# Autodesk Inventor assembly: Платформа_сборка - новая
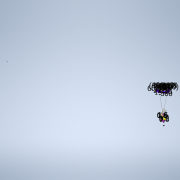
[picture p0: Inventor's stored thumbnail of the model, 180x180]
Saved by Autodesk Inventor 2020 (Build 240168000, 168)
## iProperties
Created: 2022-02-23
Part Number: Платформа_сборка - новая
Document SubType Name: Assembly
Designer: Dell
Author: Dell
## Documents named in this file (24)
- C:\Users\air13\Documents\3D\уборка\Face 2.0 full\2\Платформа_сборка - новая.iam
- C:\Users\air13\Documents\OnStage\20.05\Smile20.05VLI\Платформа_сборка_Женя\Нижний_круг_платформа.ipt
- C:\Users\air13\Documents\OnStage\20.05\Smile20.05VLI\Платформа_сборка_Женя\Крепление_мотора1_платформа.ipt
- C:\Users\air13\Documents\OnStage\20.05\Smile20.05VLI\Платформа_сборка_Женя\Крепление_мотора2_платформа.ipt
- C:\Users\air13\Documents\OnStage\20.05\Smile20.05VLI\Платформа_сборка_Женя\Крепление_мотора3_платформа.ipt
- C:\Users\air13\Documents\OnStage\20.05\Smile20.05VLI\Второй этаж\Разметка новых деталей на I этаже.ipt
- C:\Users\air13\Documents\OnStage\20.05\Smile20.05VLI\Второй этаж\Верхняя платформа.ipt
- C:\Users\air13\Documents\OnStage\20.05\Smile20.05VLI\Второй этаж\Боковой профиль.ipt
- C:\Users\air13\Documents\OnStage\20.05\Smile20.05VLI\Второй этаж\Задний профиль.ipt
- C:\Users\air13\Documents\3D\уборка\Face 2.0 full\2\шея2,0.ipt
- C:\Users\air13\Documents\OnStage\Крепление для мотора.ipt
- C:\Users\air13\Documents\OnStage\Механизм поднятия ботинка\Мотор Gekko MR25-098 без оси.ipt
- C:\Users\air13\Documents\OnStage\Механизм поднятия ботинка\Ось мотора Gekko MR25-098.ipt
- C:\Users\air13\Documents\OnStage\Механизм поднятия ботинка\Диск_для ботинка.ipt
- C:\Users\air13\Documents\OnStage\Механизм поднятия ботинка\Подшипник 604z.ipt
- C:\Users\air13\Documents\OnStage\Механизм поднятия ботинка\Поднимающая балка.ipt
- C:\Users\air13\Documents\OnStage\Механизм поднятия ботинка\Крепление_на мотор_для_диска_для ботинок.ipt
- C:\Users\air13\Documents\OnStage\Механизм поднятия ботинка\Крепление для_мотора_для руки.ipt
- C:\Users\air13\Documents\OnStage\Модель_движителя_марионеточной_опоры\Шестерня_small — копия.ipt
- C:\Users\air13\Documents\OnStage\Модель_движителя_марионеточной_опоры\Шестерня_small.ipt
- C:\Users\air13\Documents\OnStage\Модель_движителя_марионеточной_опоры\Паз_прямой_квадрат.ipt
- C:\Users\air13\Documents\OnStage\Модель_движителя_марионеточной_опоры\Шестерня_vРРО.ipt
- C:\Users\air13\Documents\OnStage\Модель_движителя_марионеточной_опоры\Проставка.ipt
- C:\Users\air13\Documents\3D\уборка\Face 2.0 full\2\ПереПереСборка лица.iam
## Components (35 placed, 22 different names)
1. Нижний_круг_платформа:1 — Угол:1, Заподлицо:1, Совмещение:1, Совмещение:2, Совмещение:3, Совмещение:5, Заподлицо:3, Совмещение:6, Заподлицо:4, Заподлицо:5, Заподлицо:6, Угол:2, Совмещение:11, Угол:3, Угол:4, Касательность:1, Совмещение:21, Совмещение:22, Совмещение:23
2. Разметка новых деталей на I этаже:1
3. Верхняя платформа:1 — Совмещение:7, Угол:2, Совмещение:8, Совмещение:9, Заподлицо:7, Совмещение:24, Совмещение:25, Угол:5, Совмещение:40, Совмещение:41, Совмещение:42, Угол:6, Совмещение:46, Совмещение:47, Совмещение:48, Совмещение:51, Совмещение:52, Совмещение:53, Совмещение:55
4. Боковой профиль:1 — Совмещение:11, Совмещение:18, Совмещение:19, Заподлицо:7, Совмещение:31
5. шея2,0:1 — Угол:3, Совмещение:13, Совмещение:19, Касательность:2, Совмещение:23, Совмещение:31, Совмещение:59, Совмещение:60
6. Задний профиль:1 — Касательность:2, Совмещение:20, Совмещение:21, Совмещение:22
7. Крепление для мотора:1 — Совмещение:24, Совмещение:25, Угол:5, Совмещение:26
8. Мотор Gekko MR25-098 без оси:1 — Совмещение:26, С поворотом:1
9. Ось мотора Gekko MR25-098:1 — С поворотом:1, С поворотом:3
10. Диск_для ботинка:1 — Совмещение:27, С поворотом:4, Совмещение:30
11. Поднимающая балка:1 — Совмещение:28, Заподлицо:8
12. Крепление_на мотор_для_диска_для ботинок:1 — С поворотом:3, Совмещение:27, Совмещение:30
13. Подшипник 604z:1 — С поворотом:4, Совмещение:28, Заподлицо:8
14. Крепление для мотора:2 — Цилиндрический:1, Совмещение:47, Совмещение:48, Совмещение:54
15. Мотор Gekko MR25-098 без оси:2 — Цилиндрический:1, С поворотом:5
16. Цилиндрическое зубчатое зацепление2:1 — Совмещение:35, Совмещение:36, Совмещение:37, Совмещение:38, Совмещение:39, Совмещение:45, Совмещение:46
17. Цилиндрическое зубчатое зацепление2:2 — Совмещение:38, Совмещение:39, Совмещение:45
18. Крепление для_мотора_для руки:1 — Цилиндрический:2, Совмещение:35, Совмещение:36, Совмещение:37
19. Ось мотора Gekko MR25-098:2 — С поворотом:5, Цилиндрический:2
20. Паз_прямой_квадрат:1 — Совмещение:40, Совмещение:41, Совмещение:42, Совмещение:43, Совмещение:44
21. Шестерня_vРРО:1 — Угол:6, Совмещение:43, Совмещение:44
22. Проставка:1 — Совмещение:51, Совмещение:52, Совмещение:53, Совмещение:54, Совмещение:55
23. ПереПереСборка лица:1 [sub-assembly] — Совмещение:59, Совмещение:60
24. Крепление_мотора1_платформа:1
25. Крепление_мотора1_платформа:2
26. Крепление_мотора1_платформа:3 — Угол:1, Заподлицо:1, Совмещение:1, Совмещение:2, Совмещение:4, Заподлицо:2
27. Крепление_мотора1_платформа:4
28. Крепление_мотора2_платформа:1 — Совмещение:5, Заподлицо:3, Совмещение:6
29. Крепление_мотора2_платформа:2
30. Крепление_мотора2_платформа:3
31. Крепление_мотора2_платформа:4
32. Крепление_мотора3_платформа:1 — Совмещение:3, Совмещение:4, Заподлицо:2
33. Крепление_мотора3_платформа:2
34. Крепление_мотора3_платформа:3
35. Крепление_мотора3_платформа:4
## Component patterns: (4 elements, first: Крепление_мотора1_платформа:1), (4 elements, first: Крепление_мотора2_платформа:1), (4 elements, first: Крепление_мотора3_платформа:1)
## Relationships (67: Mate 45, Flush 8, Angle 6, RevoluteJoint 4, Tangent 2, CylindricalJoint 2)
- Угол:1 [Angle] (0 deg): Нижний_круг_платформа:1 ↔ Крепление_мотора1_платформа:3
- Заподлицо:1 [Flush]: Нижний_круг_платформа:1 ↔ Крепление_мотора1_платформа:3
- Совмещение:1 [Mate]: Нижний_круг_платформа:1 ↔ Крепление_мотора1_платформа:3
- Совмещение:2 [Mate]: Нижний_круг_платформа:1 ↔ Крепление_мотора1_платформа:3
- Совмещение:3 [Mate]: Нижний_круг_платформа:1 ↔ Крепление_мотора3_платформа:1
- Совмещение:4 [Mate]: Крепление_мотора1_платформа:3 ↔ Крепление_мотора3_платформа:1
- Заподлицо:2 [Flush]: Крепление_мотора1_платформа:3 ↔ Крепление_мотора3_платформа:1
- Совмещение:5 [Mate]: Нижний_круг_платформа:1 ↔ Крепление_мотора2_платформа:1
- Заподлицо:3 [Flush]: Нижний_круг_платформа:1 ↔ Крепление_мотора2_платформа:1
- Совмещение:6 [Mate]: Нижний_круг_платформа:1 ↔ Крепление_мотора2_платформа:1
- Заподлицо:4 [Flush]: Нижний_круг_платформа:1
- Заподлицо:5 [Flush]: Нижний_круг_платформа:1
- Заподлицо:6 [Flush]: Нижний_круг_платформа:1
- Совмещение:7 [Mate]: Верхняя платформа:1
- Угол:2 [Angle] (0 deg): Нижний_круг_платформа:1 ↔ Верхняя платформа:1
- Совмещение:8 [Mate]: Верхняя платформа:1
- Совмещение:9 [Mate]: Верхняя платформа:1
- Совмещение:11 [Mate]: Нижний_круг_платформа:1 ↔ Боковой профиль:1
- Угол:3 [Angle] (180 deg): Нижний_круг_платформа:1 ↔ шея2,0:1
- Совмещение:13 [Mate]: шея2,0:1
- Угол:4 [Angle] (0 deg): Нижний_круг_платформа:1
- Касательность:1 [Tangent]: Нижний_круг_платформа:1
- Совмещение:18 [Mate]: Боковой профиль:1
- Совмещение:19 [Mate]: Боковой профиль:1 ↔ шея2,0:1
- Заподлицо:7 [Flush]: Верхняя платформа:1 ↔ Боковой профиль:1
- Касательность:2 [Tangent]: шея2,0:1 ↔ Задний профиль:1
- Совмещение:20 [Mate]: Задний профиль:1
- Совмещение:21 [Mate]: Нижний_круг_платформа:1 ↔ Задний профиль:1
- Совмещение:22 [Mate]: Нижний_круг_платформа:1 ↔ Задний профиль:1
- Совмещение:23 [Mate] (1035 mm): Нижний_круг_платформа:1 ↔ шея2,0:1
- Совмещение:24 [Mate]: Верхняя платформа:1 ↔ Крепление для мотора:1
- Совмещение:25 [Mate]: Верхняя платформа:1 ↔ Крепление для мотора:1
- Угол:5 [Angle] (0 deg): Верхняя платформа:1 ↔ Крепление для мотора:1
- Совмещение:26 [Mate]: Крепление для мотора:1 ↔ Мотор Gekko MR25-098 без оси:1
- С поворотом:1 [RevoluteJoint]: Мотор Gekko MR25-098 без оси:1 ↔ Ось мотора Gekko MR25-098:1
- С поворотом:3 [RevoluteJoint]: Ось мотора Gekko MR25-098:1 ↔ Крепление_на мотор_для_диска_для ботинок:1
- Совмещение:27 [Mate]: Диск_для ботинка:1 ↔ Крепление_на мотор_для_диска_для ботинок:1
- С поворотом:4 [RevoluteJoint] (-4 mm): Диск_для ботинка:1 ↔ Подшипник 604z:1
- Совмещение:28 [Mate]: Поднимающая балка:1 ↔ Подшипник 604z:1
- Совмещение:30 [Mate]: Диск_для ботинка:1 ↔ Крепление_на мотор_для_диска_для ботинок:1
- Заподлицо:8 [Flush]: Поднимающая балка:1 ↔ Подшипник 604z:1
- Совмещение:31 [Mate]: Боковой профиль:1 ↔ шея2,0:1
- Цилиндрический:1 [CylindricalJoint]: Крепление для мотора:2 ↔ Мотор Gekko MR25-098 без оси:2
- С поворотом:5 [RevoluteJoint]: Мотор Gekko MR25-098 без оси:2 ↔ Ось мотора Gekko MR25-098:2
- Цилиндрический:2 [CylindricalJoint]: Крепление для_мотора_для руки:1 ↔ Ось мотора Gekko MR25-098:2
- Совмещение:35 [Mate]: Цилиндрическое зубчатое зацепление2:1 ↔ Крепление для_мотора_для руки:1
- Совмещение:36 [Mate]: Цилиндрическое зубчатое зацепление2:1 ↔ Крепление для_мотора_для руки:1
- Совмещение:37 [Mate]: Цилиндрическое зубчатое зацепление2:1 ↔ Крепление для_мотора_для руки:1
- Совмещение:38 [Mate]: Цилиндрическое зубчатое зацепление2:1 ↔ Цилиндрическое зубчатое зацепление2:2
- Совмещение:39 [Mate]: Цилиндрическое зубчатое зацепление2:1 ↔ Цилиндрическое зубчатое зацепление2:2
- Совмещение:40 [Mate]: Верхняя платформа:1 ↔ Паз_прямой_квадрат:1
- Совмещение:41 [Mate]: Верхняя платформа:1 ↔ Паз_прямой_квадрат:1
- Совмещение:42 [Mate]: Верхняя платформа:1 ↔ Паз_прямой_квадрат:1
- Угол:6 [Angle] (0 deg): Верхняя платформа:1 ↔ Шестерня_vРРО:1
- Совмещение:43 [Mate] (1 mm): Паз_прямой_квадрат:1 ↔ Шестерня_vРРО:1
- Совмещение:44 [Mate]: Паз_прямой_квадрат:1 ↔ Шестерня_vРРО:1
- Совмещение:45 [Mate]: Цилиндрическое зубчатое зацепление2:1 ↔ Цилиндрическое зубчатое зацепление2:2
- Совмещение:46 [Mate] (5 mm): Верхняя платформа:1 ↔ Цилиндрическое зубчатое зацепление2:1
- Совмещение:47 [Mate]: Верхняя платформа:1 ↔ Крепление для мотора:2
- Совмещение:48 [Mate]: Верхняя платформа:1 ↔ Крепление для мотора:2
- Совмещение:51 [Mate]: Верхняя платформа:1 ↔ Проставка:1
- Совмещение:52 [Mate]: Верхняя платформа:1 ↔ Проставка:1
- Совмещение:53 [Mate]: Верхняя платформа:1 ↔ Проставка:1
- Совмещение:54 [Mate]: Крепление для мотора:2 ↔ Проставка:1
- Совмещение:55 [Mate]: Верхняя платформа:1 ↔ Проставка:1
- Совмещение:59 [Mate]: шея2,0:1 ↔ ПереПереСборка лица:1
- Совмещение:60 [Mate]: шея2,0:1 ↔ ПереПереСборка лица:1
